# Autodesk Inventor assembly: aluminium engine v2
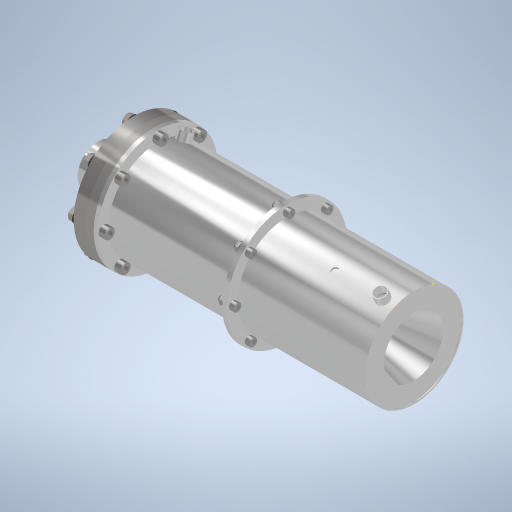
[picture p0: Inventor's stored thumbnail of the model, 512x512]
Saved by Autodesk Inventor 2023 (Build 270158000, 158)
## iProperties
Created: 2022-09-29
Part Number: aluminium engine v2
Document SubType Name: Assembly
Designer: station
Author: station
## Documents named in this file (12)
- C:\Users\station\Documents\Project\Liquid-engine-cooling-system\design files\ethanol engine 6\Aluminium engine v2\aluminium engine v2.iam
- C:\Users\station\Documents\Project\Liquid-engine-cooling-system\design files\ethanol engine 6\Aluminium engine v2\aluminium engine v2.ipt
- C:\Users\station\Documents\Project\Liquid-engine-cooling-system\design files\ethanol engine 6\Aluminium engine v2\stainless steel space.ipt
- C:\Users\station\Documents\Project\Liquid-engine-cooling-system\design files\ethanol engine 6\Aluminium engine v2\aluminium outer wall - front.ipt
- C:\Users\station\Documents\Project\Liquid-engine-cooling-system\design files\ethanol engine 6\Aluminium engine v2\aluminium outer wall back.ipt
- C:\Users\station\Documents\Project\Liquid-engine-cooling-system\design files\injector_design_files\WANYOIKE.iam
- C:\Users\station\Documents\Inventor\Content Center Files\R2023\en-US\ISO 4762(2)\ISO 4762 - M8 x 40ISO.ipt
- C:\Users\station\Documents\Inventor\Content Center Files\R2023\en-US\ISO 7091\ISO 7091 - ST 8 - 100 HV.ipt
- C:\Users\station\Documents\Inventor\Content Center Files\R2023\en-US\ISO 4032(2)\ISO 4032 - M8 - ISO.ipt
- C:\Users\station\Documents\Inventor\Content Center Files\R2023\en-US\ISO 4762(2)\ISO 4762 - M6 x 16ISO.ipt
- C:\Users\station\Documents\Inventor\Content Center Files\R2023\en-US\ISO 7091\ISO 7091 - ST 6 - 100 HV.ipt
- C:\Users\station\Documents\Inventor\Content Center Files\R2023\en-US\ISO 4032(2)\ISO 4032 - M6 - ISO.ipt
## Components (53 placed, 11 different names)
1. aluminium engine v2:1 — Mate:1, Mate:2, Mate:6, Mate:7, Mate:10, Mate:12, Mate:13
2. stainless steel space:1 — Mate:1, Mate:2, Mate:5
3. aluminium outer wall - front:1 — Mate:6, Mate:7, Mate:8, Mate:9, Mate:10, Mate:11, Mate:14, Mate:15, Mate:16, Mate:17, Mate:18, Mate:19, Mate:20, Mate:21, Mate:22, Mate:23, Mate:24, Mate:25, Mate:26, Mate:27, Mate:28, Mate:29, Mate:30, Mate:32, Mate:34, Mate:36, Mate:38, Mate:40, Mate:42, Mate:44, Mate:63, Mate:65, Mate:67, Mate:69, Mate:71, Mate:73, Mate:75, Mate:77
4. aluminium outer wall back:1 — Mate:5, Mate:8, Mate:11, Mate:46, Mate:47, Mate:48, Mate:49, Mate:50, Mate:51, Mate:52, Mate:53, Mate:54, Mate:55, Mate:56, Mate:57, Mate:58, Mate:59, Mate:60, Mate:61, Mate:62, Mate:64, Mate:66, Mate:68, Mate:70, Mate:72, Mate:74, Mate:76
5. WANYOIKE:1 [sub-assembly] — Mate:9, Mate:12, Mate:13, Mate:31, Mate:33, Mate:35, Mate:37, Mate:39, Mate:41, Mate:43, Mate:45
6. ISO 4762 M8 x 40:1 — Mate:14, Mate:15
7. ISO 7091 ST 8 - 100 HV:1 — Mate:30, Mate:31, Insert:1
8. ISO 4032 M8:1 — Insert:1
9. ISO 4762 M8 x 40:2 — Mate:16, Mate:17
10. ISO 4762 M8 x 40:3 — Mate:18, Mate:19
11. ISO 4762 M8 x 40:4 — Mate:20, Mate:21
12. ISO 4762 M8 x 40:5 — Mate:22, Mate:23
13. ISO 4762 M8 x 40:6 — Mate:24, Mate:25
14. ISO 4762 M8 x 40:7 — Mate:26, Mate:27
15. ISO 4762 M8 x 40:8 — Mate:28, Mate:29
16. ISO 7091 ST 8 - 100 HV:2 — Mate:32, Mate:33, Insert:2
17. ISO 7091 ST 8 - 100 HV:3 — Mate:34, Mate:35, Insert:3
18. ISO 7091 ST 8 - 100 HV:4 — Mate:36, Mate:37, Insert:4
19. ISO 7091 ST 8 - 100 HV:5 — Mate:38, Mate:39, Insert:5
20. ISO 7091 ST 8 - 100 HV:6 — Mate:40, Mate:41, Insert:6
21. ISO 7091 ST 8 - 100 HV:7 — Mate:42, Mate:43, Insert:7
22. ISO 7091 ST 8 - 100 HV:8 — Mate:44, Mate:45, Insert:8
23. ISO 4032 M8:2 — Insert:2
24. ISO 4032 M8:3 — Insert:3
25. ISO 4032 M8:4 — Insert:4
26. ISO 4032 M8:5 — Insert:5
27. ISO 4032 M8:6 — Insert:6
28. ISO 4032 M8:7 — Insert:7
29. ISO 4032 M8:8 — Insert:8
30. ISO 4762 M6 x 16:1 — Mate:46, Mate:47
31. ISO 7091 ST 6 - 100 HV:1 — Mate:62, Mate:63, Insert:9
32. ISO 4032 M6:1 — Insert:9
33. ISO 4762 M6 x 16:2 — Mate:48, Mate:49
34. ISO 4762 M6 x 16:3 — Mate:50, Mate:51
35. ISO 4762 M6 x 16:4 — Mate:52, Mate:53
36. ISO 4762 M6 x 16:5 — Mate:54, Mate:55
37. ISO 4762 M6 x 16:6 — Mate:56, Mate:57
38. ISO 4762 M6 x 16:7 — Mate:58, Mate:59
39. ISO 4762 M6 x 16:8 — Mate:60, Mate:61
40. ISO 7091 ST 6 - 100 HV:2 — Mate:64, Mate:65, Insert:10
41. ISO 7091 ST 6 - 100 HV:3 — Mate:66, Mate:67, Insert:11
42. ISO 7091 ST 6 - 100 HV:4 — Mate:68, Mate:69, Insert:12
43. ISO 7091 ST 6 - 100 HV:5 — Mate:70, Mate:71, Insert:13
44. ISO 7091 ST 6 - 100 HV:6 — Mate:72, Mate:73, Insert:14
45. ISO 7091 ST 6 - 100 HV:7 — Mate:74, Mate:75, Insert:15
46. ISO 7091 ST 6 - 100 HV:8 — Mate:76, Mate:77, Insert:16
47. ISO 4032 M6:2 — Insert:10
48. ISO 4032 M6:3 — Insert:11
49. ISO 4032 M6:4 — Insert:12
50. ISO 4032 M6:5 — Insert:13
51. ISO 4032 M6:6 — Insert:14
52. ISO 4032 M6:7 — Insert:15
53. ISO 4032 M6:8 — Insert:16
## Relationships (91: Mate 75, Insert 16)
- Mate:1: aluminium engine v2:1 ↔ stainless steel space:1
- Mate:2 (13.716 mm): aluminium engine v2:1 ↔ stainless steel space:1
- Mate:5: stainless steel space:1 ↔ aluminium outer wall back:1
- Mate:6: aluminium engine v2:1 ↔ aluminium outer wall - front:1
- Mate:7: aluminium engine v2:1 ↔ aluminium outer wall - front:1
- Mate:8: aluminium outer wall - front:1 ↔ aluminium outer wall back:1
- Mate:9: aluminium outer wall - front:1 ↔ WANYOIKE:1
- Mate:10: aluminium engine v2:1 ↔ aluminium outer wall - front:1
- Mate:11: aluminium outer wall - front:1 ↔ aluminium outer wall back:1
- Mate:12: aluminium engine v2:1 ↔ WANYOIKE:1
- Mate:13: aluminium engine v2:1 ↔ WANYOIKE:1
- Mate:14: aluminium outer wall - front:1 ↔ ISO 4762 M8 x 40:1
- Mate:15: aluminium outer wall - front:1 ↔ ISO 4762 M8 x 40:1
- Mate:16: aluminium outer wall - front:1 ↔ ISO 4762 M8 x 40:2
- Mate:17: aluminium outer wall - front:1 ↔ ISO 4762 M8 x 40:2
- Mate:18: aluminium outer wall - front:1 ↔ ISO 4762 M8 x 40:3
- Mate:19: aluminium outer wall - front:1 ↔ ISO 4762 M8 x 40:3
- Mate:20: aluminium outer wall - front:1 ↔ ISO 4762 M8 x 40:4
- Mate:21: aluminium outer wall - front:1 ↔ ISO 4762 M8 x 40:4
- Mate:22: aluminium outer wall - front:1 ↔ ISO 4762 M8 x 40:5
- Mate:23: aluminium outer wall - front:1 ↔ ISO 4762 M8 x 40:5
- Mate:24: aluminium outer wall - front:1 ↔ ISO 4762 M8 x 40:6
- Mate:25: aluminium outer wall - front:1 ↔ ISO 4762 M8 x 40:6
- Mate:26: aluminium outer wall - front:1 ↔ ISO 4762 M8 x 40:7
- Mate:27: aluminium outer wall - front:1 ↔ ISO 4762 M8 x 40:7
- Mate:28: aluminium outer wall - front:1 ↔ ISO 4762 M8 x 40:8
- Mate:29: aluminium outer wall - front:1 ↔ ISO 4762 M8 x 40:8
- Mate:30: aluminium outer wall - front:1 ↔ ISO 7091 ST 8 - 100 HV:1
- Mate:31: WANYOIKE:1 ↔ ISO 7091 ST 8 - 100 HV:1
- Mate:32: aluminium outer wall - front:1 ↔ ISO 7091 ST 8 - 100 HV:2
- Mate:33: WANYOIKE:1 ↔ ISO 7091 ST 8 - 100 HV:2
- Mate:34: aluminium outer wall - front:1 ↔ ISO 7091 ST 8 - 100 HV:3
- Mate:35: WANYOIKE:1 ↔ ISO 7091 ST 8 - 100 HV:3
- Mate:36: aluminium outer wall - front:1 ↔ ISO 7091 ST 8 - 100 HV:4
- Mate:37: WANYOIKE:1 ↔ ISO 7091 ST 8 - 100 HV:4
- Mate:38: aluminium outer wall - front:1 ↔ ISO 7091 ST 8 - 100 HV:5
- Mate:39: WANYOIKE:1 ↔ ISO 7091 ST 8 - 100 HV:5
- Mate:40: aluminium outer wall - front:1 ↔ ISO 7091 ST 8 - 100 HV:6
- Mate:41: WANYOIKE:1 ↔ ISO 7091 ST 8 - 100 HV:6
- Mate:42: aluminium outer wall - front:1 ↔ ISO 7091 ST 8 - 100 HV:7
- Mate:43: WANYOIKE:1 ↔ ISO 7091 ST 8 - 100 HV:7
- Mate:44: aluminium outer wall - front:1 ↔ ISO 7091 ST 8 - 100 HV:8
- Mate:45: WANYOIKE:1 ↔ ISO 7091 ST 8 - 100 HV:8
- Insert:1: ISO 7091 ST 8 - 100 HV:1 ↔ ISO 4032 M8:1
- Insert:2: ISO 7091 ST 8 - 100 HV:2 ↔ ISO 4032 M8:2
- Insert:3: ISO 7091 ST 8 - 100 HV:3 ↔ ISO 4032 M8:3
- Insert:4: ISO 7091 ST 8 - 100 HV:4 ↔ ISO 4032 M8:4
- Insert:5: ISO 7091 ST 8 - 100 HV:5 ↔ ISO 4032 M8:5
- Insert:6: ISO 7091 ST 8 - 100 HV:6 ↔ ISO 4032 M8:6
- Insert:7: ISO 7091 ST 8 - 100 HV:7 ↔ ISO 4032 M8:7
- Insert:8: ISO 7091 ST 8 - 100 HV:8 ↔ ISO 4032 M8:8
- Mate:46: aluminium outer wall back:1 ↔ ISO 4762 M6 x 16:1
- Mate:47: aluminium outer wall back:1 ↔ ISO 4762 M6 x 16:1
- Mate:48: aluminium outer wall back:1 ↔ ISO 4762 M6 x 16:2
- Mate:49: aluminium outer wall back:1 ↔ ISO 4762 M6 x 16:2
- Mate:50: aluminium outer wall back:1 ↔ ISO 4762 M6 x 16:3
- Mate:51: aluminium outer wall back:1 ↔ ISO 4762 M6 x 16:3
- Mate:52: aluminium outer wall back:1 ↔ ISO 4762 M6 x 16:4
- Mate:53: aluminium outer wall back:1 ↔ ISO 4762 M6 x 16:4
- Mate:54: aluminium outer wall back:1 ↔ ISO 4762 M6 x 16:5
- Mate:55: aluminium outer wall back:1 ↔ ISO 4762 M6 x 16:5
- Mate:56: aluminium outer wall back:1 ↔ ISO 4762 M6 x 16:6
- Mate:57: aluminium outer wall back:1 ↔ ISO 4762 M6 x 16:6
- Mate:58: aluminium outer wall back:1 ↔ ISO 4762 M6 x 16:7
- Mate:59: aluminium outer wall back:1 ↔ ISO 4762 M6 x 16:7
- Mate:60: aluminium outer wall back:1 ↔ ISO 4762 M6 x 16:8
- Mate:61: aluminium outer wall back:1 ↔ ISO 4762 M6 x 16:8
- Mate:62: aluminium outer wall back:1 ↔ ISO 7091 ST 6 - 100 HV:1
- Mate:63: aluminium outer wall - front:1 ↔ ISO 7091 ST 6 - 100 HV:1
- Mate:64: aluminium outer wall back:1 ↔ ISO 7091 ST 6 - 100 HV:2
- Mate:65: aluminium outer wall - front:1 ↔ ISO 7091 ST 6 - 100 HV:2
- Mate:66: aluminium outer wall back:1 ↔ ISO 7091 ST 6 - 100 HV:3
- Mate:67: aluminium outer wall - front:1 ↔ ISO 7091 ST 6 - 100 HV:3
- Mate:68: aluminium outer wall back:1 ↔ ISO 7091 ST 6 - 100 HV:4
- Mate:69: aluminium outer wall - front:1 ↔ ISO 7091 ST 6 - 100 HV:4
- Mate:70: aluminium outer wall back:1 ↔ ISO 7091 ST 6 - 100 HV:5
- Mate:71: aluminium outer wall - front:1 ↔ ISO 7091 ST 6 - 100 HV:5
- Mate:72: aluminium outer wall back:1 ↔ ISO 7091 ST 6 - 100 HV:6
- Mate:73: aluminium outer wall - front:1 ↔ ISO 7091 ST 6 - 100 HV:6
- Mate:74: aluminium outer wall back:1 ↔ ISO 7091 ST 6 - 100 HV:7
- Mate:75: aluminium outer wall - front:1 ↔ ISO 7091 ST 6 - 100 HV:7
- Mate:76: aluminium outer wall back:1 ↔ ISO 7091 ST 6 - 100 HV:8
- Mate:77: aluminium outer wall - front:1 ↔ ISO 7091 ST 6 - 100 HV:8
- Insert:9: ISO 7091 ST 6 - 100 HV:1 ↔ ISO 4032 M6:1
- Insert:10: ISO 7091 ST 6 - 100 HV:2 ↔ ISO 4032 M6:2
- Insert:11: ISO 7091 ST 6 - 100 HV:3 ↔ ISO 4032 M6:3
- Insert:12: ISO 7091 ST 6 - 100 HV:4 ↔ ISO 4032 M6:4
- Insert:13: ISO 7091 ST 6 - 100 HV:5 ↔ ISO 4032 M6:5
- Insert:14: ISO 7091 ST 6 - 100 HV:6 ↔ ISO 4032 M6:6
- Insert:15: ISO 7091 ST 6 - 100 HV:7 ↔ ISO 4032 M6:7
- Insert:16: ISO 7091 ST 6 - 100 HV:8 ↔ ISO 4032 M6:8
